# Autodesk Inventor assembly: antenna_holder
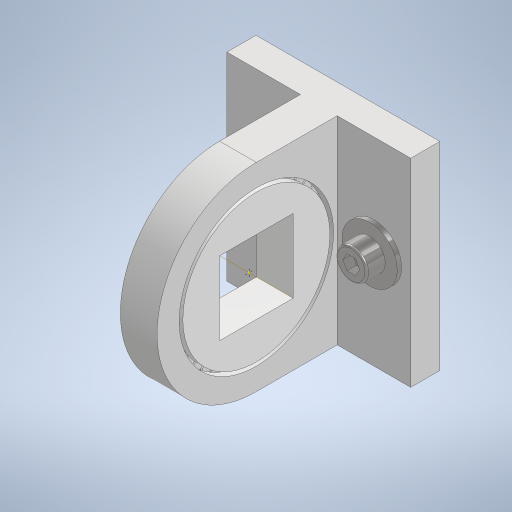
[picture p0: Inventor's stored thumbnail of the model, 512x512]
Saved by Autodesk Inventor 2024 (Build 280153000, 153)
## iProperties
Created: 2025-12-27
Part Number: antenna_holder
Document SubType Name: Assembly
Designer: schar
Author: schar
## Documents named in this file (7)
- C:\Users\schar\Desktop\projectBlueprint\AMSTS\hardware\antenna_holder.iam
- C:\Users\schar\Desktop\projectBlueprint\AMSTS\hardware\antenna_rad.ipt
- C:\Users\schar\Desktop\projectBlueprint\AMSTS\hardware\antenna_rad_outter.ipt
- C:\Users\schar\Documents\Inventor\Content Center Files\R2024\en-US\ISO 4762(1)\DIN EN ISO 4762 - M5 x 16.ipt
- C:\Users\schar\Documents\Inventor\Content Center Files\R2024\en-US\DIN 9021\DIN 9021 - 5,3.ipt
- C:\Users\schar\Desktop\projectBlueprint\AMSTS\hardware\tnut_m5_2020.ipt
- C:\Users\schar\Desktop\projectBlueprint\AMSTS\hardware\bearing_stifts_antenna.ipt
## Components (9 placed, 6 different names)
1. antenna_rad:1 — Mate:1, Flush:1, Mate:10
2. antenna_rad_outter:1 — Mate:1, Flush:1, Mate:2, Mate:3, Mate:4, Mate:5, Mate:8, Mate:9, Rigid:1, Rigid:2, Mate:11
3. DIN EN ISO 4762 M5 x 16:1 — Mate:6, Mate:9
4. DIN EN ISO 4762 M5 x 16:2 — Mate:7, Mate:8
5. DIN 9021 5,3:1 — Mate:2, Mate:5, Mate:6
6. DIN 9021 5,3:2 — Mate:3, Mate:4, Mate:7
7. tnut_m5_2020:1 — Rigid:2
8. tnut_m5_2020:2 — Rigid:1
9. bearing_stifts_antenna:1 — Mate:10, Mate:11
## Relationships (14: Mate 11, WeldJoint 2, Flush 1)
- Mate:1: antenna_rad:1 ↔ antenna_rad_outter:1
- Flush:1: antenna_rad:1 ↔ antenna_rad_outter:1
- Mate:2: antenna_rad_outter:1 ↔ DIN 9021 5,3:1
- Mate:3: antenna_rad_outter:1 ↔ DIN 9021 5,3:2
- Mate:4: antenna_rad_outter:1 ↔ DIN 9021 5,3:2
- Mate:5: antenna_rad_outter:1 ↔ DIN 9021 5,3:1
- Mate:6: DIN EN ISO 4762 M5 x 16:1 ↔ DIN 9021 5,3:1
- Mate:7: DIN EN ISO 4762 M5 x 16:2 ↔ DIN 9021 5,3:2
- Mate:8: antenna_rad_outter:1 ↔ DIN EN ISO 4762 M5 x 16:2
- Mate:9: antenna_rad_outter:1 ↔ DIN EN ISO 4762 M5 x 16:1
- Rigid:1 [WeldJoint] (-0.159 mm): antenna_rad_outter:1 ↔ tnut_m5_2020:2
- Rigid:2 [WeldJoint] (-0.159 mm): antenna_rad_outter:1 ↔ tnut_m5_2020:1
- Mate:10: antenna_rad:1 ↔ bearing_stifts_antenna:1
- Mate:11: antenna_rad_outter:1 ↔ bearing_stifts_antenna:1
